# Autodesk Inventor assembly: Application_Fluorescence_Microscope_Infinity_Berlin_v3
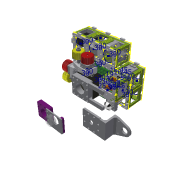
[picture p0: Inventor's stored thumbnail of the model, 180x180]
Saved by Autodesk Inventor 2022 (Build 260153000, 153)
## iProperties
Created: 2019-07-16
Part Number: Application_Fluorescence_Microscope_Infinity_Berlin_v3
Document SubType Name: Assembly
Designer: marsikovabarbora
Mass: 572.046 g
Surface Area: 3822.31 cm^2
Volume: 517.299 cm^3
Density: 1.10583 g/cm^3
Author: marsikovabarbora
## Documents named in this file (11)
- C:\Users\diederichbenedict\Dropbox\Dokumente\Promotion\PROJECTS\UC2\02_CAD\INVENTOR\uc2_v3\Application_Fluorescence_Microscope_Infinity_Berlin_v3.iam
- C:\Users\diederichbenedict\Dropbox\Dokumente\Promotion\PROJECTS\UC2\02_CAD\INVENTOR\uc2_v3\Assembly_Cube_Lens_holder_165mm_v3.iam
- C:\Users\diederichbenedict\Dropbox\Dokumente\Promotion\PROJECTS\UC2\02_CAD\INVENTOR\uc2_v3\Assembly_Cube_Dichroic_Beamsplitter_25x35_v3.iam
- C:\Users\diederichbenedict\Dropbox\Dokumente\Promotion\PROJECTS\UC2\02_CAD\INVENTOR\uc2_v3\Assembly_Cube_AlliedVision_Alvium_v3.iam
- C:\Users\diederichbenedict\Dropbox\Dokumente\Promotion\PROJECTS\UC2\02_CAD\INVENTOR\uc2_v3\Assembly_Cube_Laser_Block_v3.iam
- C:\Users\diederichbenedict\Dropbox\Dokumente\Promotion\PROJECTS\UC2\02_CAD\INVENTOR\uc2_v3\10_Base_puzzle_v3.ipt
- C:\Users\diederichbenedict\Dropbox\Dokumente\Promotion\PROJECTS\UC2\02_CAD\INVENTOR\uc2_v3\Assembly_Cube_Kinematic_Mirrormount_Thorlabs_45_v3.iam
- C:\Users\diederichbenedict\Dropbox\Dokumente\Promotion\PROJECTS\UC2\02_CAD\INVENTOR\uc2_v3\00_Microscope_Objective.ipt
- C:\Users\diederichbenedict\Dropbox\Dokumente\Promotion\PROJECTS\UC2\02_CAD\INVENTOR\uc2_v3\Assembly_Cube_Mirror_Thorlabs_v3.iam
- C:\Users\diederichbenedict\Dropbox\Dokumente\Promotion\PROJECTS\UC2\02_CAD\INVENTOR\uc2_v3\Assembly_XY_stage_with_motors_v3.iam
- C:\Users\diederichbenedict\Dropbox\Dokumente\Promotion\PROJECTS\UC2\02_CAD\INVENTOR\uc2_v3\Assembly_Cube_Z_Focus_MGN_NEMA_v3.iam
## Components (35 placed, 10 different names)
1. Assembly_Cube_Mirror_Thorlabs_v3:1 [sub-assembly] — Insert:9, Mate:13
2. Assembly_Cube_Lens_holder_165mm_v3:1 [sub-assembly] — Insert:2
3. Assembly_Cube_AlliedVision_Alvium_v3:1 [sub-assembly] — Insert:4
4. Assembly_Cube_Lens_holder_165mm_v3:2 [sub-assembly] — Insert:3
5. Assembly_Cube_Kinematic_Mirrormount_Thorlabs_45_v3:2 [sub-assembly] — Insert:5
6. Assembly_XY_stage_with_motors_v3:1 [sub-assembly] — Mate:11, Flush:4, Mate:13
7. 00_Microscope_Objective:1 — Einfügen:17
8. 10_Base_puzzle_v3:13 — Mate:3, Flush:2, Flush:3, Insert:9
9. Assembly_Cube_Dichroic_Beamsplitter_25x35_v3:1 [sub-assembly] — Einfügen:13
10. Assembly_Cube_Kinematic_Mirrormount_Thorlabs_45_v3:3 [sub-assembly] — Einfügen:14
11. Assembly_Cube_Z_Focus_MGN_NEMA_v3:1 [sub-assembly] — Einfügen:15, Einfügen:17
12. Assembly_Cube_Mirror_Thorlabs_v3:2 [sub-assembly] — Einfügen:16
13. Assembly_Cube_Laser_Block_v3:1 [sub-assembly] — Einfügen:18
14. 10_Base_puzzle_v3:1 — Mate:1, Mate:2, Flush:1, Insert:5
15. 10_Base_puzzle_v3:2 — Insert:2
16. 10_Base_puzzle_v3:3
17. 10_Base_puzzle_v3:4 — Mate:3, Flush:2, Flush:3
18. 10_Base_puzzle_v3:5 — Insert:4
19. 10_Base_puzzle_v3:6
20. 10_Base_puzzle_v3:7
21. 10_Base_puzzle_v3:8 — Insert:3
22. 10_Base_puzzle_v3:9
23. 10_Base_puzzle_v3:27
24. 10_Base_puzzle_v3:28
25. 10_Base_puzzle_v3:29 — Flush:4, Einfügen:13, Passend:14, Fluchtend:5, Fluchtend:6
26. 10_Base_puzzle_v3:30 — Mate:11
27. 10_Base_puzzle_v3:31
28. 10_Base_puzzle_v3:32
29. 10_Base_puzzle_v3:33 — Einfügen:18
30. 10_Base_puzzle_v3:34
31. 10_Base_puzzle_v3:35 — Einfügen:14
32. 10_Base_puzzle_v3:36 — Passend:14, Fluchtend:5, Fluchtend:6
33. 10_Base_puzzle_v3:37
34. 10_Base_puzzle_v3:38 — Einfügen:16
35. 10_Base_puzzle_v3:39 — Einfügen:15
## Component patterns: (2 elements), (2 elements), (9 elements, first: 10_Base_puzzle_v3:1), Component Pattern 1:2 (9 elements), (2 elements, first: 10_Base_puzzle_v3:36), Komponentenanordnung 7:2 (2 elements)
## Relationships (23: Insert 11, Mate 6, Flush 6)
- Mate:1: 10_Base_puzzle_v3:1
- Mate:2: 10_Base_puzzle_v3:1
- Flush:1: 10_Base_puzzle_v3:1
- Mate:3: 10_Base_puzzle_v3:13 ↔ 10_Base_puzzle_v3:4
- Flush:2: 10_Base_puzzle_v3:13 ↔ 10_Base_puzzle_v3:4
- Flush:3: 10_Base_puzzle_v3:13 ↔ 10_Base_puzzle_v3:4
- Insert:2: Assembly_Cube_Lens_holder_165mm_v3:1 ↔ 10_Base_puzzle_v3:2
- Insert:3: Assembly_Cube_Lens_holder_165mm_v3:2 ↔ 10_Base_puzzle_v3:8
- Insert:4: Assembly_Cube_AlliedVision_Alvium_v3:1 ↔ 10_Base_puzzle_v3:5
- Insert:5: Assembly_Cube_Kinematic_Mirrormount_Thorlabs_45_v3:2 ↔ 10_Base_puzzle_v3:1
- Insert:9: Assembly_Cube_Mirror_Thorlabs_v3:1 ↔ 10_Base_puzzle_v3:13
- Mate:11: Assembly_XY_stage_with_motors_v3:1 ↔ 10_Base_puzzle_v3:30
- Flush:4: Assembly_XY_stage_with_motors_v3:1 ↔ 10_Base_puzzle_v3:29
- Mate:13: Assembly_Cube_Mirror_Thorlabs_v3:1 ↔ Assembly_XY_stage_with_motors_v3:1
- Einfügen:13 [Insert]: Assembly_Cube_Dichroic_Beamsplitter_25x35_v3:1 ↔ 10_Base_puzzle_v3:29
- Einfügen:14 [Insert]: Assembly_Cube_Kinematic_Mirrormount_Thorlabs_45_v3:3 ↔ 10_Base_puzzle_v3:35
- Passend:14 [Mate]: 10_Base_puzzle_v3:29 ↔ 10_Base_puzzle_v3:36
- Fluchtend:5 [Flush]: 10_Base_puzzle_v3:29 ↔ 10_Base_puzzle_v3:36
- Fluchtend:6 [Flush]: 10_Base_puzzle_v3:29 ↔ 10_Base_puzzle_v3:36
- Einfügen:15 [Insert]: Assembly_Cube_Z_Focus_MGN_NEMA_v3:1 ↔ 10_Base_puzzle_v3:39
- Einfügen:16 [Insert]: Assembly_Cube_Mirror_Thorlabs_v3:2 ↔ 10_Base_puzzle_v3:38
- Einfügen:17 [Insert] (-10 mm): 00_Microscope_Objective:1 ↔ Assembly_Cube_Z_Focus_MGN_NEMA_v3:1
- Einfügen:18 [Insert]: Assembly_Cube_Laser_Block_v3:1 ↔ 10_Base_puzzle_v3:33
